# Autodesk Inventor assembly: Clamex Joint114
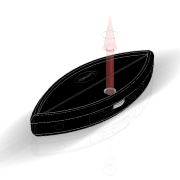
[picture p0: Inventor's stored thumbnail of the model, 180x180]
Saved by Autodesk Inventor 2024 (Build 280153000, 153)
## iProperties
RuleStatus: InUse
Created: 2023-01-31
Part Number: Clamex Joint114
Document SubType Name: Assembly
Designer: sauliusd
Author: sauliusd
## Documents named in this file (3)
- C:\W4INV 2024 Design\PROJECTS\Samples\Macro DEMO\5 Lamello ClamexTest Box\Test Lamelo Box.iam Smart Hardware\Clamex Joint114\Clamex Joint114.iam
- C:\W4INV 2024 Design\PROJECTS\Samples\Macro DEMO\5 Lamello ClamexTest Box\Test Lamelo Box.iam Smart Hardware\Clamex Joint114\Clamex Joint11400.ipt
- C:\W4INV 2024 Design\LIBRARY\Fixed joints\Lamello Clamex P-14\Clamex P-14 Connector.iam
## Components (3 placed, 3 different names)
1. @Skeleton — Mate:1, Flush:1, Flush:3
2. Clamex P-14 Lammelo — Mate:1, Flush:1
3. Clamex P-14 Connector:2 [sub-assembly]
## Component patterns: (2 elements, first: Clamex P-14 Lammelo)
## Relationships (3: Flush 2, Mate 1)
- Mate:1: @Skeleton ↔ Clamex P-14 Lammelo
- Flush:1: @Skeleton ↔ Clamex P-14 Lammelo
- Flush:3: @Skeleton
## Named parameters: ContactPatchWidth = 381 mm, ContactPatchHeight = 21.939 mm, ConnectionAngle = 120 deg, NestledBoardT = 19 mm, PillarBoardT = 19 mm, MinDistFromSide = 50 mm, SideDist1 = 60 mm, MaxDistBetween = 480 mm, SideDist2 = 60 mm, MaxDistFromSide = 180 mm, ShiftY = 0 mm
